# Autodesk Inventor assembly: FullMidFrame
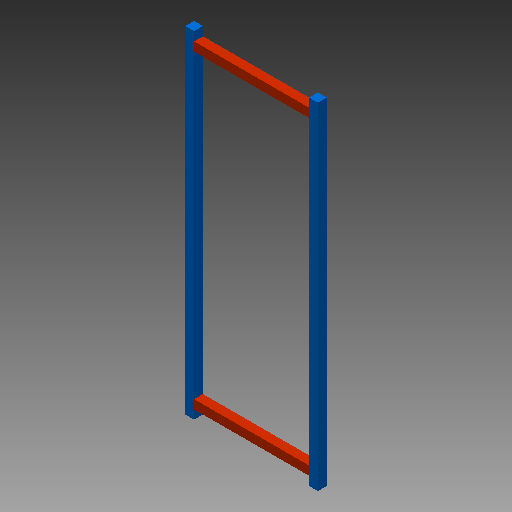
[picture p0: Inventor's stored thumbnail of the model, 512x512]
Saved by Autodesk Inventor 2019 (Build 230136000, 136)
## iProperties
Created: 2019-01-09
Part Number: FullMidFrame
Document SubType Name: Assembly
Designer: james
Author: james
## Documents named in this file (3)
- F:\JimsDesign\2019CHS4089\FullMidFrame.iam
- F:\JimsDesign\2019CHS4089\CrossBeam.ipt
- F:\JimsDesign\2019CHS4089\MidBeam.ipt
## Components (4 placed, 2 different names)
1. CrossBeam:1 — Mate:1, Flush:1, Flush:2, Mate:2, Flush:3, Flush:4
2. CrossBeam:2 — Mate:3, Flush:5, Flush:6
3. MidBeam:1 — Mate:1, Flush:1, Flush:2, Mate:3, Flush:5, Flush:6
4. MidBeam:2 — Mate:2, Flush:3, Flush:4
## Relationships (9: Flush 6, Mate 3)
- Mate:1: CrossBeam:1 ↔ MidBeam:1
- Flush:1: CrossBeam:1 ↔ MidBeam:1
- Flush:2 (-25.4 mm): CrossBeam:1 ↔ MidBeam:1
- Mate:2: CrossBeam:1 ↔ MidBeam:2
- Flush:3: CrossBeam:1 ↔ MidBeam:2
- Flush:4 (25.4 mm): CrossBeam:1 ↔ MidBeam:2
- Mate:3: CrossBeam:2 ↔ MidBeam:1
- Flush:5 (25.4 mm): CrossBeam:2 ↔ MidBeam:1
- Flush:6: CrossBeam:2 ↔ MidBeam:1
